# Autodesk Inventor assembly: 3.25 Omni AS, Square_MIR
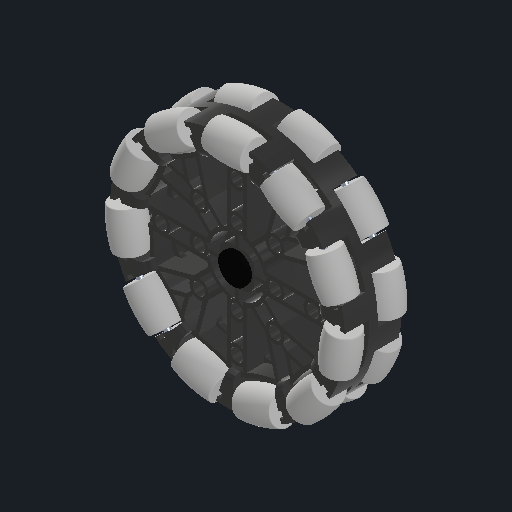
[picture p0: Inventor's stored thumbnail of the model, 512x512]
Saved by Autodesk Inventor 2023 (Build 270158000, 158)
## iProperties
Created: 2022-08-02
Part Number: 3.25 Omni AS, Square_MIR
Document SubType Name: Assembly
Designer: Windows Macbook
Author: ylu12
## Documents named in this file (3)
- C:\Users\Windows Macbook\Desktop\VRC-SPIN-UP\Inventor\Motion\Wheels\Omni Wheel\3.25 Omni AS, Square_MIR.iam
- C:\Users\Windows Macbook\Desktop\VRC-SPIN-UP\Inventor\Motion\Wheels\Reference Files\3.25 Omni Antistatic_MIR.ipt
- C:\Users\Windows Macbook\Desktop\VRC-SPIN-UP\Inventor\Motion\Insert Square_MIR3.ipt
## Components (3 placed, 2 different names)
1. 3.25 Omni Antistatic_MIR:1 — Mate:12, Mate:11, Flush:6
2. Insert Square_MIR3:1 — Flush:11, Flush:10, Mate:17
3. Insert Square_MIR3:2 — Angle:1, Mate:18, Flush:11, Flush:10, Flush:9
## Relationships (9: Mate 4, Flush 4, Angle 1)
- Mate:12: 3.25 Omni Antistatic_MIR:1
- Mate:11: 3.25 Omni Antistatic_MIR:1
- Flush:6: 3.25 Omni Antistatic_MIR:1
- Angle:1 (0 deg): Insert Square_MIR3:2
- Mate:18: Insert Square_MIR3:2
- Flush:11: Insert Square_MIR3:1 ↔ Insert Square_MIR3:2
- Flush:10: Insert Square_MIR3:1 ↔ Insert Square_MIR3:2
- Flush:9 [Mate] (6.35 mm): Insert Square_MIR3:2
- Mate:17 [Flush] (6.35 mm): Insert Square_MIR3:1
